# Autodesk Inventor assembly: Assembly1
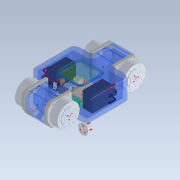
[picture p0: Inventor's stored thumbnail of the model, 180x180]
Saved by Autodesk Inventor 2020 (Build 240168000, 168)
## iProperties
Created: 2021-01-08
Part Number: Assembly1
Document SubType Name: Assembly
Designer: DELL
Author: DELL
## Documents named in this file (10)
- F:\SoftRobot2.0\FlexipodHardware2.0\FlexipodHardware\Flexipod2.0\robot_2021_1_8\Assembly1.iam
- F:\SoftRobot2.0\FlexipodHardware2.0\FlexipodHardware\Flexipod2.0\robot_2021_1_8\body.ipt
- F:\SoftRobot2.0\FlexipodHardware2.0\FlexipodHardware\Flexipod2.0\RMD_X6_stator.ipt
- F:\SoftRobot2.0\FlexipodHardware2.0\FlexipodHardware\Flexipod2.0\RMD_X6_rotor.ipt
- F:\SoftRobot2.0\FlexipodHardware2.0\FlexipodHardware\Flexipod2.0\robot_2021_1_8\hip_link_front.ipt
- F:\SoftRobot2.0\FlexipodHardware2.0\FlexipodHardware\Flexipod2.0\robot_2021_1_8\hip_link_front_mirror.ipt
- F:\SoftRobot2.0\FlexipodHardware2.0\FlexipodHardware\Flexipod2.0\robot_2021_1_8\hip_link_back.ipt
- F:\SoftRobot2.0\FlexipodHardware2.0\FlexipodHardware\Flexipod2.0\robot_2021_1_8\hip_link_back_mirror.ipt
- F:\SoftRobot2.0\FlexipodHardware2.0\FlexipodHardware\Flexipod2.0\Jetson nano v2- Inventor\Jetson_Nano_Dev_Kit_3D_b01.iam
- F:\SoftRobot2.0\FlexipodHardware2.0\FlexipodHardware\Flexipod2.0\battery_6s_1550_ovonic.ipt
## Components (18 placed, 9 different names)
1. body:1 — Flush:1, Mate:1, Flush:2, Mate:6, Mate:7, Mate:8, Mate:9, Mate:10, Mate:11, Mate:12, Mate:13, Mate:14, Mate:15, Mate:16, Mate:17
2. RMD_X6_stator:1 — Mate:2, Flush:3, Mate:6, Mate:7, Mate:8, Mate:19
3. RMD_X6_rotor:1 — Mate:2, Flush:3, Mate:18, Mate:20
4. RMD_X6_stator:2 — Mate:9, Mate:10, Mate:11, Mate:28
5. RMD_X6_rotor:2 — Mate:27, Mate:29
6. RMD_X6_stator:3 — Mate:15, Mate:16, Mate:17, Mate:21
7. RMD_X6_rotor:3 — Mate:22, Mate:23
8. RMD_X6_stator:4 — Mate:12, Mate:13, Mate:14, Mate:25
9. RMD_X6_rotor:4 — Mate:24, Mate:26
10. hip_link_front:1 — Mate:18, Mate:19, Mate:20, Mate:38, Mate:39, Mate:40
11. hip_link_front_mirror:1 — Mate:21, Mate:22, Mate:23
12. hip_link_back:1 — Mate:24, Mate:25, Mate:26
13. hip_link_back_mirror:1 — Mate:27, Mate:28, Mate:29
14. RMD_X6_stator:5 — Mate:38, Mate:39, Mate:40
15. RMD_X6_rotor:5
16. Jetson_Nano_Dev_Kit_3D_b01:1 [sub-assembly]
17. battery_6s_1550_ovonic:1
18. battery_6s_1550_ovonic:2
## Relationships (40: Mate 33, Flush 7)
- Flush:1: body:1
- Mate:1: body:1
- Flush:2: body:1
- Mate:2: RMD_X6_stator:1 ↔ RMD_X6_rotor:1
- Flush:3 (-3 mm): RMD_X6_stator:1 ↔ RMD_X6_rotor:1
- [Mate]: RMD_X6_stator:2 ↔ RMD_X6_rotor:2
- [Flush] (-3 mm): RMD_X6_stator:2 ↔ RMD_X6_rotor:2
- [Mate]: RMD_X6_stator:3 ↔ RMD_X6_rotor:3
- [Flush] (-3 mm): RMD_X6_stator:3 ↔ RMD_X6_rotor:3
- [Mate]: RMD_X6_stator:4 ↔ RMD_X6_rotor:4
- [Flush] (-3 mm): RMD_X6_stator:4 ↔ RMD_X6_rotor:4
- Mate:6: body:1 ↔ RMD_X6_stator:1
- Mate:7: body:1 ↔ RMD_X6_stator:1
- Mate:8: body:1 ↔ RMD_X6_stator:1
- Mate:9: body:1 ↔ RMD_X6_stator:2
- Mate:10: body:1 ↔ RMD_X6_stator:2
- Mate:11: body:1 ↔ RMD_X6_stator:2
- Mate:12: body:1 ↔ RMD_X6_stator:4
- Mate:13: body:1 ↔ RMD_X6_stator:4
- Mate:14: body:1 ↔ RMD_X6_stator:4
- Mate:15: body:1 ↔ RMD_X6_stator:3
- Mate:16: body:1 ↔ RMD_X6_stator:3
- Mate:17: body:1 ↔ RMD_X6_stator:3
- Mate:18: RMD_X6_rotor:1 ↔ hip_link_front:1
- Mate:19: RMD_X6_stator:1 ↔ hip_link_front:1
- Mate:20: RMD_X6_rotor:1 ↔ hip_link_front:1
- Mate:21: RMD_X6_stator:3 ↔ hip_link_front_mirror:1
- Mate:22: RMD_X6_rotor:3 ↔ hip_link_front_mirror:1
- Mate:23: RMD_X6_rotor:3 ↔ hip_link_front_mirror:1
- Mate:24: RMD_X6_rotor:4 ↔ hip_link_back:1
- Mate:25: RMD_X6_stator:4 ↔ hip_link_back:1
- Mate:26: RMD_X6_rotor:4 ↔ hip_link_back:1
- Mate:27: RMD_X6_rotor:2 ↔ hip_link_back_mirror:1
- Mate:28: RMD_X6_stator:2 ↔ hip_link_back_mirror:1
- Mate:29: RMD_X6_rotor:2 ↔ hip_link_back_mirror:1
- [Mate]: RMD_X6_stator:5 ↔ RMD_X6_rotor:5
- [Flush] (-3 mm): RMD_X6_stator:5 ↔ RMD_X6_rotor:5
- Mate:38: hip_link_front:1 ↔ RMD_X6_stator:5
- Mate:39: hip_link_front:1 ↔ RMD_X6_stator:5
- Mate:40: hip_link_front:1 ↔ RMD_X6_stator:5
## Named parameters: d5_d3 = 0 mm, d6_d4 = -3 mm, d7_d3 = 0 mm, d8_d4 = -3 mm, d9_d3 = 0 mm, d10_d4 = -3 mm, d35_d3 = 0 mm, d36_d4 = -3 mm
